# Autodesk Inventor assembly: assemblybattery
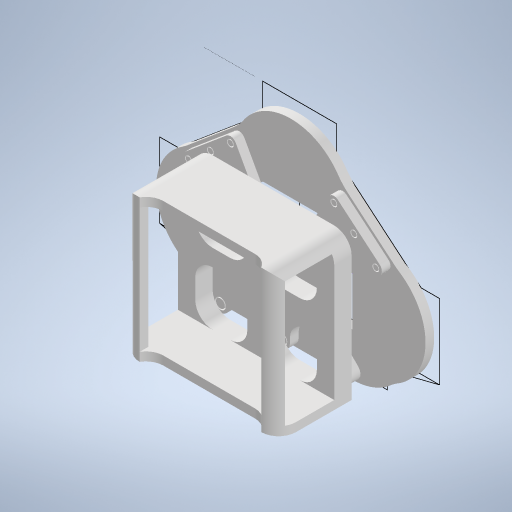
[picture p0: Inventor's stored thumbnail of the model, 512x512]
Saved by Autodesk Inventor 2023 (Build 270158000, 158)
## iProperties
Created: 2023-02-09
Part Number: assemblybattery
Document SubType Name: Assembly
Designer: zayda
Author: zayda
## Documents named in this file (4)
- C:\Users\zayda\Documents\assemblybattery.iam
- C:\Users\zayda\Documents\batteryclip.ipt
- C:\Users\zayda\Documents\batteryclip2.ipt
- C:\Users\zayda\Documents\batteryclip3.ipt
## Components (3 placed, 3 different names)
1. batteryclip:1 — Mate:1, Mate:2
2. batteryclip2:1 — Mate:1, Mate:2, Mate:3, Mate:4, Mate:5
3. batteryclip3:1 — Mate:3, Mate:4, Mate:5
## Relationships (5: Mate 5)
- Mate:1: batteryclip:1 ↔ batteryclip2:1
- Mate:2: batteryclip:1 ↔ batteryclip2:1
- Mate:3: batteryclip2:1 ↔ batteryclip3:1
- Mate:4: batteryclip2:1 ↔ batteryclip3:1
- Mate:5: batteryclip2:1 ↔ batteryclip3:1
